# Autodesk Inventor assembly: 00_052_LOADCELL_CONTACT_R1
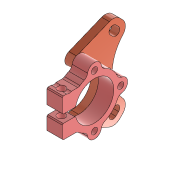
[picture p0: Inventor's stored thumbnail of the model, 180x180]
Saved by Autodesk Inventor 2021.2 (Build 252289000, 289)
## iProperties
Created: 2021-03-07
Part Number: 00_052_LOADCELL_CONTACT_R1
Document SubType Name: Assembly
Designer: y6tada
Author: y6tada
## Documents named in this file (5)
- C:\Workspace\HaptHexa\Hardware\Inventor\00_052_LOADCELL_CONTACT_R1.iam
- C:\Workspace\HaptHexa\Hardware\Inventor\16_022_TIBIA_PIPE_CLAMPER_R1.ipt
- C:\Workspace\HaptHexa\Hardware\Inventor\16_014_SENSOR_LOD_CON_R1.ipt
- C:\Workspace\HaptHexa\Hardware\Inventor\10_053_CAP_BOLT_M2X10_R1.ipt
- C:\Workspace\HaptHexa\Hardware\Inventor\10_047_LOW_HEAD_SCREW_M2X5_R1.ipt
## Components (6 placed, 4 different names)
1. 16_022_TIBIA_PIPE_CLAMPER_R1:1 — Mate:2, Insert:4
2. 16_014_SENSOR_LOD_CON_R1:1 — Mate:2, Insert:1, Insert:2, Insert:3
3. 10_053_CAP_BOLT_M2X10_R1:1 — Insert:4
4. 10_047_LOW_HEAD_SCREW_M2X5_R1:1 — Insert:1
5. 10_047_LOW_HEAD_SCREW_M2X5_R1:2 — Insert:2
6. 10_047_LOW_HEAD_SCREW_M2X5_R1:3 — Insert:3
## Relationships (7: Insert 4, Mate 2, Flush 1)
- [Flush]: 16_022_TIBIA_PIPE_CLAMPER_R1:1 ↔ 16_014_SENSOR_LOD_CON_R1:1
- [Mate]: 16_022_TIBIA_PIPE_CLAMPER_R1:1 ↔ 16_014_SENSOR_LOD_CON_R1:1
- Mate:2: 16_022_TIBIA_PIPE_CLAMPER_R1:1 ↔ 16_014_SENSOR_LOD_CON_R1:1
- Insert:1: 16_014_SENSOR_LOD_CON_R1:1 ↔ 10_047_LOW_HEAD_SCREW_M2X5_R1:1
- Insert:2: 16_014_SENSOR_LOD_CON_R1:1 ↔ 10_047_LOW_HEAD_SCREW_M2X5_R1:2
- Insert:3: 16_014_SENSOR_LOD_CON_R1:1 ↔ 10_047_LOW_HEAD_SCREW_M2X5_R1:3
- Insert:4: 16_022_TIBIA_PIPE_CLAMPER_R1:1 ↔ 10_053_CAP_BOLT_M2X10_R1:1
